# Autodesk Inventor assembly: Beam Splitter
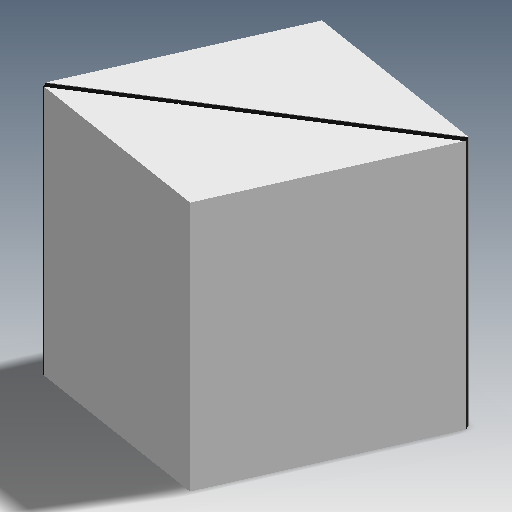
[picture p0: Inventor's stored thumbnail of the model, 512x512]
Saved by Autodesk Inventor 2026 (Build 300175050, 175E)
## iProperties
Created: 2025-08-02
Part Number: Beam Splitter
Document SubType Name: Assembly
Designer: aman0
Author: aman0
## Documents named in this file (3)
- D:\Academics\Projects\Physics Enabled Raytracer\Code\Models\Beam Splitter.iam
- D:\Academics\Projects\Physics Enabled Raytracer\Code\Models\Beamsplittertransparent.ipt
- D:\Academics\Projects\Physics Enabled Raytracer\Code\Models\BeamsplitterReflect.ipt
## Components (2 placed, 2 different names)
1. Beamsplittertransparent:1 — Mate:1, Flush:1
2. BeamsplitterReflect:1 — Mate:1, Flush:1
## Relationships (2: Mate 1, Flush 1)
- Mate:1: Beamsplittertransparent:1 ↔ BeamsplitterReflect:1
- Flush:1: Beamsplittertransparent:1 ↔ BeamsplitterReflect:1
